# Autodesk Inventor assembly: linear-unit
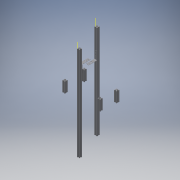
[picture p0: Inventor's stored thumbnail of the model, 180x180]
Saved by Autodesk Inventor 2016 (Build 200138000, 138)
## iProperties
Created: 2015-10-07
Part Number: linear-unit
Document SubType Name: Assembly
Designer: Thomas
Author: Thomas
## Documents named in this file (5)
- C:\Thomas\Projects\make-it-move\cad-linear\cad\linear-unit.iam
- C:\Thomas\Projects\make-it-move\cad-linear\cad\assets\maker-beam-300x10x10mm.ipt
- C:\Thomas\Projects\make-it-move\cad-linear\cad\assets\maker-beam-60x10x10mm.ipt
- C:\Thomas\Projects\make-it-move\cad-linear\cad\assets\maker-beam-40x10x10mm.ipt
- C:\Thomas\Projects\make-it-move\cad-linear\cad\assets\maker-beam-corner.ipt
## Components (10 placed, 4 different names)
1. maker-beam-300x10x10mm:1 — Mate:1, Mate:2, Mate:9, Mate:10
2. maker-beam-60x10x10mm:1 — Mate:1, Mate:3, Mate:4
3. maker-beam-60x10x10mm:2 — Mate:6, Mate:8
4. maker-beam-300x10x10mm:2 — Mate:5, Mate:8, Mate:11
5. maker-beam-40x10x10mm:1
6. maker-beam-40x10x10mm:2
7. maker-beam-40x10x10mm:3
8. maker-beam-40x10x10mm:4
9. maker-beam-corner:1 — Mate:11
10. maker-beam-corner:2 — Mate:9, Mate:10
## Relationships (11: Mate 11)
- Mate:1: maker-beam-300x10x10mm:1 ↔ maker-beam-60x10x10mm:1
- Mate:2: maker-beam-300x10x10mm:1
- Mate:3: maker-beam-60x10x10mm:1
- Mate:4: maker-beam-60x10x10mm:1
- Mate:5: maker-beam-300x10x10mm:2
- Mate:6: maker-beam-60x10x10mm:2
- Mate:7
- Mate:8: maker-beam-60x10x10mm:2 ↔ maker-beam-300x10x10mm:2
- Mate:9: maker-beam-300x10x10mm:1 ↔ maker-beam-corner:2
- Mate:10: maker-beam-300x10x10mm:1 ↔ maker-beam-corner:2
- Mate:11: maker-beam-300x10x10mm:2 ↔ maker-beam-corner:1
